# Autodesk Inventor assembly: Assembly2
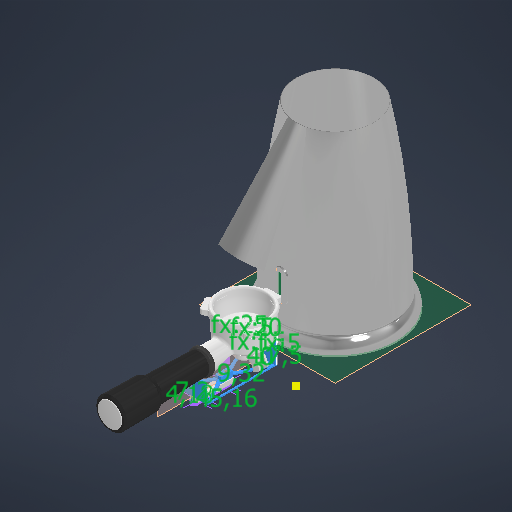
[picture p0: Inventor's stored thumbnail of the model, 512x512]
Saved by Autodesk Inventor 2026 (Build 300175000, 175)
## iProperties
Created: 2025-04-29
Part Number: Assembly2
Document SubType Name: Assembly
Designer: Paul Juschitz
Author: Paul Juschitz
## Documents named in this file (5)
- C:\Users\Paul Juschitz\Documents\private\m5_GBW_mod\M5_GBW_mod\CAD\Assembly2.iam
- C:\Users\Paul Juschitz\Documents\private\m5_GBW_mod\M5_GBW_mod\CAD\holder_assembly_2.iam
- C:\Users\Paul Juschitz\Documents\Inventor\Content Center Files\R2026\en-US\BS EN ISO 7046-2 H\BS EN ISO 7046-2 H - M3x10 - 8.8 - H1.ipt
- C:\Users\Paul Juschitz\Documents\private\m5_GBW_mod\M5_GBW_mod\CAD\load_cell.ipt
- C:\Users\Paul Juschitz\Documents\private\m5_GBW_mod\M5_GBW_mod\CAD\m2m_shell.ipt
## Components (5 placed, 4 different names)
1. holder_assembly_2:1 [sub-assembly] — Mate:1, Mate:2, Mate:3, Mate:4, Angle:1, Mate:6, Mate:7
2. BS EN ISO 7046-2 H M3x10 - 8.8 - H1:1 — Mate:1, Mate:2
3. BS EN ISO 7046-2 H M3x10 - 8.8 - H1:2 — Mate:3, Mate:4, Mate:5
4. load_cell:1 — Mate:5, Angle:1, Mate:6
5. m2m_shell:1 — Mate:7
## Relationships (8: Mate 7, Angle 1)
- Mate:1: holder_assembly_2:1 ↔ BS EN ISO 7046-2 H M3x10 - 8.8 - H1:1
- Mate:2: holder_assembly_2:1 ↔ BS EN ISO 7046-2 H M3x10 - 8.8 - H1:1
- Mate:3: holder_assembly_2:1 ↔ BS EN ISO 7046-2 H M3x10 - 8.8 - H1:2
- Mate:4: holder_assembly_2:1 ↔ BS EN ISO 7046-2 H M3x10 - 8.8 - H1:2
- Mate:5: BS EN ISO 7046-2 H M3x10 - 8.8 - H1:2 ↔ load_cell:1
- Angle:1 (0 deg): holder_assembly_2:1 ↔ load_cell:1
- Mate:6: holder_assembly_2:1 ↔ load_cell:1
- Mate:7: holder_assembly_2:1 ↔ m2m_shell:1
